# Autodesk Inventor assembly: CameraUnit
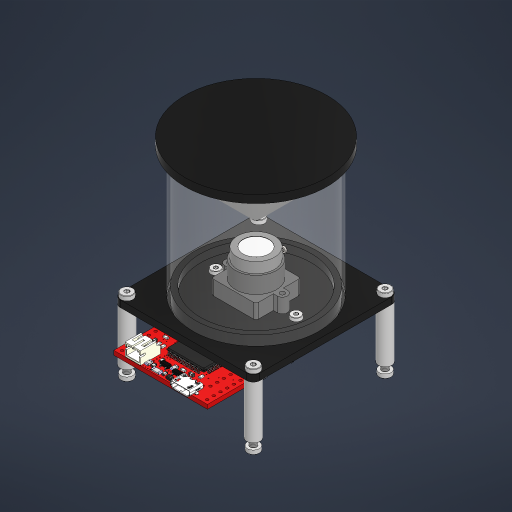
[picture p0: Inventor's stored thumbnail of the model, 512x512]
Saved by Autodesk Inventor 2024.2 (Build 282272000, 272)
## iProperties
Created: 2023-12-21
Part Number: CameraUnit
Document SubType Name: Assembly
Designer: Hanaoka
Author: Hanaoka
## Documents named in this file (8)
- G:\共有ドライブ\reRo\05_個人\hanaoka\inventor\CameraUnit\CameraUnit.iam
- G:\共有ドライブ\reRo\05_個人\hanaoka\inventor\CameraUnit\Camera_pipe.ipt
- G:\共有ドライブ\reRo\05_個人\hanaoka\inventor\CameraUnit\Camera_mirror.ipt
- G:\共有ドライブ\reRo\05_個人\hanaoka\inventor\CameraUnit\OpenMV_H7\OpenMV_H7.iam
- G:\共有ドライブ\reRo\05_個人\hanaoka\inventor\Screw\M2xL6\M2x6.ipt
- G:\共有ドライブ\reRo\05_個人\hanaoka\inventor\Spacer\Spacer_M2.6x20.ipt
- G:\共有ドライブ\reRo\05_個人\hanaoka\inventor\CameraUnit\Camera_Mount.ipt
- G:\共有ドライブ\reRo\05_個人\hanaoka\inventor\Screw\M2.6x8\M2.6x8.ipt
## Components (18 placed, 7 different names)
1. Camera_pipe:1 — 挿入:2
2. Camera_mirror:1 — 挿入:2
3. OpenMV_H7:1 [sub-assembly] — フラッシュ:1
4. M2x6:1
5. M2x6:2
6. Spacer_M2.6x20:1 — 挿入:8
7. Spacer_M2.6x20:2 — 挿入:9
8. Spacer_M2.6x20:3 — 挿入:10
9. Spacer_M2.6x20:4 — 挿入:7
10. Camera_Mount:1 — フラッシュ:1, 挿入:3, 挿入:4, 挿入:5, 挿入:6
11. M2.6x8:1 — 挿入:6
12. M2.6x8:2 — 挿入:5
13. M2.6x8:3 — 挿入:3
14. M2.6x8:4 — 挿入:4
15. M2.6x8:5 — 挿入:7
16. M2.6x8:6 — 挿入:10
17. M2.6x8:7 — 挿入:9
18. M2.6x8:8 — 挿入:8
## Relationships (10: Insert 9, Flush 1)
- 挿入:2 [Insert]: Camera_pipe:1 ↔ Camera_mirror:1
- フラッシュ:1 [Flush]: OpenMV_H7:1 ↔ Camera_Mount:1
- 挿入:3 [Insert]: Camera_Mount:1 ↔ M2.6x8:3
- 挿入:4 [Insert]: Camera_Mount:1 ↔ M2.6x8:4
- 挿入:5 [Insert]: Camera_Mount:1 ↔ M2.6x8:2
- 挿入:6 [Insert]: Camera_Mount:1 ↔ M2.6x8:1
- 挿入:7 [Insert] (2.5 mm): Spacer_M2.6x20:4 ↔ M2.6x8:5
- 挿入:8 [Insert] (2.5 mm): Spacer_M2.6x20:1 ↔ M2.6x8:8
- 挿入:9 [Insert] (2.5 mm): Spacer_M2.6x20:2 ↔ M2.6x8:7
- 挿入:10 [Insert] (2.5 mm): Spacer_M2.6x20:3 ↔ M2.6x8:6
